# Autodesk Inventor assembly: bras_main
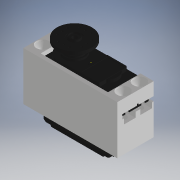
[picture p0: Inventor's stored thumbnail of the model, 180x180]
Saved by Autodesk Inventor 2020 (Build 240168000, 168)
## iProperties
Created: 2019-12-27
Part Number: bras_main
Document SubType Name: Assembly
Designer: bapti
Author: bapti
## Documents named in this file (3)
- C:\Users\bapti\Documents\EIRBOT\eirbot2020-2A\Meca\EIRBOT_sailtheworld\robot\bras\bras_main.iam
- C:\Users\bapti\Documents\EIRBOT\eirbot2020-2A\Meca\EIRBOT_sailtheworld\robot\bras\servo_holder.ipt
- C:\Users\bapti\Documents\EIRBOT\eirbot2020-2A\Meca\EIRBOT_sailtheworld\mg995\MG_996R.iam
## Components (2 placed, 2 different names)
1. servo_holder:1 — Affleurement:1, Placage:1, Affleurement:2, Placage:2, Placage:3, Placage:4
2. MG_996R:1 [sub-assembly] — Placage:2, Placage:3, Placage:4
## Relationships (6: Mate 4, Flush 2)
- Affleurement:1 [Flush]: servo_holder:1
- Placage:1 [Mate]: servo_holder:1
- Affleurement:2 [Flush]: servo_holder:1
- Placage:2 [Mate]: servo_holder:1 ↔ MG_996R:1
- Placage:3 [Mate]: servo_holder:1 ↔ MG_996R:1
- Placage:4 [Mate]: servo_holder:1 ↔ MG_996R:1
